# Autodesk Inventor assembly: 足全体
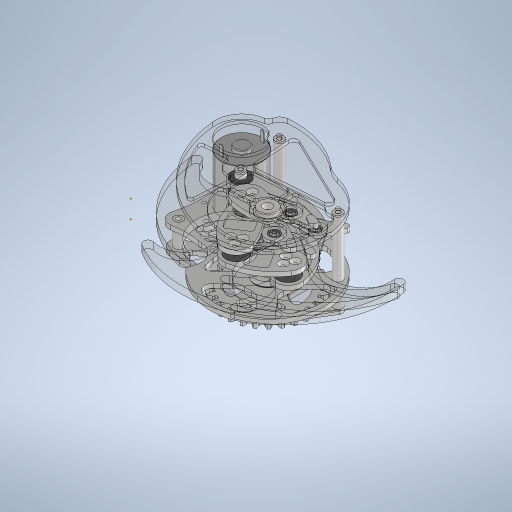
[picture p0: Inventor's stored thumbnail of the model, 512x512]
Saved by Autodesk Inventor 2023 (Build 270158000, 158)
## iProperties
Created: 2022-01-30
Part Number: 足全体
Document SubType Name: Assembly
Designer: acps
Author: acps
## Documents named in this file (3)
- C:\Users\acps\Documents\srdc\srdc_ksh\脚\足全体.iam
- C:\Users\acps\Documents\srdc\srdc_ksh\脚\足ユニット.iam
- C:\Users\acps\Documents\srdc\srdc_ksh\スペーサ\l19.ipt
## Components (2 placed, 2 different names)
1. 足ユニット:1 [sub-assembly] — Insert:8
2. l19:1 — Insert:8
## Relationships (1: Insert 1)
- Insert:8: 足ユニット:1 ↔ l19:1
